# Autodesk Inventor assembly: motorassembly
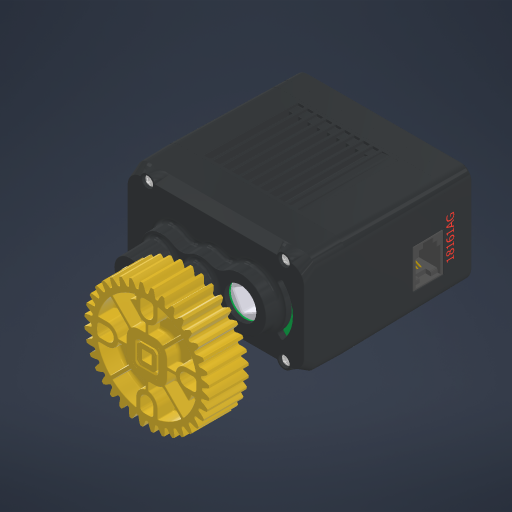
[picture p0: Inventor's stored thumbnail of the model, 512x512]
Saved by Autodesk Inventor 2023 (Build 270158000, 158)
## iProperties
Created: 2023-08-05
Part Number: motorassembly
Document SubType Name: Assembly
Designer: srbel
Author: srbel
## Documents named in this file (6)
- C:\CAD\OverUnderCAD\Drive\motorassembly.iam
- C:\CAD\OverUnderCAD\VEX-CAD-Inventor-1.4.0\Motion\Gears\HS Gear\HS 36T Gear, Square.iam
- C:\CAD\OverUnderCAD\VEX-CAD-Inventor-1.4.0\Motion\Gears\HS Gear.iam
- C:\CAD\OverUnderCAD\VEX-CAD-Inventor-1.4.0\Motion\Spacers\Spacer Nylon .313 OD\NSpacer .313 OD x .250.ipt
- C:\CAD\OverUnderCAD\VEX-CAD-Inventor-1.4.0\Motion\Spacers\Spacer Nylon .313 OD.ipt
- C:\CAD\OverUnderCAD\VEX-CAD-Inventor-1.4.0\Electronics\V5 Motor.ipt
## Components (3 placed, 3 different names)
1. HS 36T Gear, Square:1 [sub-assembly] — Insert:1
2. NSpacer .313 OD x .250:1 — Insert:1, Insert:2
3. V5 Motor:1 — Insert:2
## Relationships (2: Insert 2)
- Insert:1: HS 36T Gear, Square:1 ↔ NSpacer .313 OD x .250:1
- Insert:2 (11.0236 mm): NSpacer .313 OD x .250:1 ↔ V5 Motor:1
